# Autodesk Inventor assembly: Lift Assembly
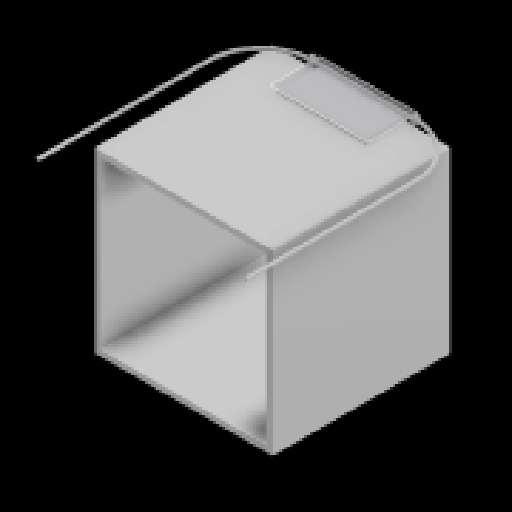
[picture p0: Inventor's stored thumbnail of the model, 512x512]
Saved by Autodesk Inventor 2025 (Build 290162000, 162)
## iProperties
Created: 2024-10-10
Part Number: Lift Assembly
Document SubType Name: Assembly
Designer: AdminForWorker
Title: Lift Assembly v1
Author: AdminForWorker
## Documents named in this file (6)
- C:\Users\Trevor\Documents\GitHub\USA-Robotic-Club-2024\assests\Lift Assembly v1\Lift Assembly.iam
- C:\Users\Trevor\Documents\GitHub\USA-Robotic-Club-2024\assests\Lift Assembly v1\ball bearing v2.iam
- C:\Users\Trevor\Documents\GitHub\USA-Robotic-Club-2024\assests\Lift Assembly v1\ball bearing Copy v1.iam
- C:\Users\Trevor\Documents\GitHub\USA-Robotic-Club-2024\assests\Lift Assembly v1\dolly lift v2.ipt
- C:\Users\Trevor\Documents\GitHub\USA-Robotic-Club-2024\assests\Lift Assembly v1\Bin v1.ipt
- C:\Users\Trevor\Documents\GitHub\USA-Robotic-Club-2024\assests\Lift Assembly v1\Part14.ipt
## Components (5 placed, 5 different names)
1. ball bearing v2:1 [sub-assembly]
2. ball bearing Copy v1:1 [sub-assembly]
3. dolly lift v2:1 — Flush:1
4. Bin v1:1
5. Part14
## Relationships (1: Flush 1)
- Flush:1 (3.175 mm): dolly lift v2:1
